# Autodesk Inventor assembly: end_casing_testfit
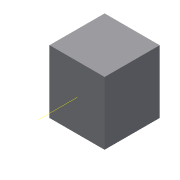
[picture p0: Inventor's stored thumbnail of the model, 180x180]
Saved by Autodesk Inventor 2017 (Build 210142000, 142)
## iProperties
Created: 2018-06-13
Part Number: end_casing_testfit
Document SubType Name: Assembly
Designer: Nic
Author: Nic
## Documents named in this file (4)
- C:\Users\Nic\Documents\Antenna\end_casing_testfit.iam
- C:\Users\Nic\Documents\Antenna\mould_end_casing_base.ipt
- C:\Users\Nic\Documents\Antenna\end_segment_v2.ipt
- C:\Users\Nic\Documents\Antenna\mould_end_casing_top.ipt
## Components (3 placed, 3 different names)
1. mould_end_casing_base:1 — Mate:1, Mate:2, Mate:3, Mate:4, Insert:1, Insert:2
2. end_segment_v2:1 — Mate:1, Mate:2, Mate:3
3. mould_end_casing_top:1 — Mate:4, Insert:1, Insert:2
## Relationships (6: Mate 4, Insert 2)
- Mate:1 (0.2 mm): mould_end_casing_base:1 ↔ end_segment_v2:1
- Mate:2 (0.5 mm): mould_end_casing_base:1 ↔ end_segment_v2:1
- Mate:3 (0.4 mm): mould_end_casing_base:1 ↔ end_segment_v2:1
- Mate:4: mould_end_casing_base:1 ↔ mould_end_casing_top:1
- Insert:1: mould_end_casing_base:1 ↔ mould_end_casing_top:1
- Insert:2: mould_end_casing_base:1 ↔ mould_end_casing_top:1
